# Autodesk Inventor assembly: Arms
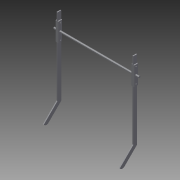
[picture p0: Inventor's stored thumbnail of the model, 180x180]
Saved by Autodesk Inventor 2013 (Build 170138000, 138)
## iProperties
Created: 2014-01-21
Part Number: Arms
Document SubType Name: Assembly
Designer: RobertB
Author: RobertB
## Documents named in this file (4)
- D:\Robotics\FRC\2014\CAD\Robot\Pickup\Arms.iam
- D:\Robotics\FRC\2014\CAD\Robot\Pickup\PickupArm.ipt
- D:\Robotics\FRC\2014\CAD\Robot\Pickup\SuperHexagon.ipt
- D:\Robotics\FRC\2014\CAD\Robot\Pickup\ArmPlate.ipt
## Components (7 placed, 3 different names)
1. PickupArm:1 — Mate:1, Flush:1, Flush:2, Flush:8, Mate:15, Mate:16, Flush:9
2. PickupArm:2 — Mate:1, Flush:1, Flush:2, Flush:4, Flush:6, Mate:12, Flush:7, Mate:13, Mate:20
3. SuperHexagon:1 — Flush:4, Mate:18, Mate:19, Mate:20, Mate:21
4. ArmPlate:1 — Flush:8, Mate:15, Mate:17
5. ArmPlate:2 — Flush:7, Mate:13, Mate:14
6. ArmPlate:3 — Mate:16, Flush:9, Mate:17, Mate:21
7. ArmPlate:4 — Flush:6, Mate:12, Mate:14, Mate:18, Mate:19
## Relationships (18: Mate 11, Flush 7)
- Mate:1 (508 mm): PickupArm:1 ↔ PickupArm:2
- Flush:1: PickupArm:1 ↔ PickupArm:2
- Flush:2: PickupArm:1 ↔ PickupArm:2
- Flush:4 (28.575 mm): PickupArm:2 ↔ SuperHexagon:1
- Flush:6: PickupArm:2 ↔ ArmPlate:4
- Mate:12: PickupArm:2 ↔ ArmPlate:4
- Flush:7: PickupArm:2 ↔ ArmPlate:2
- Mate:13: PickupArm:2 ↔ ArmPlate:2
- Mate:14: ArmPlate:2 ↔ ArmPlate:4
- Flush:8: PickupArm:1 ↔ ArmPlate:1
- Mate:15: PickupArm:1 ↔ ArmPlate:1
- Mate:16: PickupArm:1 ↔ ArmPlate:3
- Flush:9: PickupArm:1 ↔ ArmPlate:3
- Mate:17: ArmPlate:1 ↔ ArmPlate:3
- Mate:18: SuperHexagon:1 ↔ ArmPlate:4
- Mate:19: SuperHexagon:1 ↔ ArmPlate:4
- Mate:20: PickupArm:2 ↔ SuperHexagon:1
- Mate:21: SuperHexagon:1 ↔ ArmPlate:3
